# Autodesk Inventor assembly: 775pro_0_1-2inHex
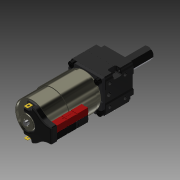
[picture p0: Inventor's stored thumbnail of the model, 180x180]
Saved by Autodesk Inventor 2021 (Build 250183000, 183)
## iProperties
Created: 2018-08-19
Part Number: 775pro_0_1-2inHex
Document SubType Name: Assembly
Designer: Rafi
Mass: 1123.04 g
Surface Area: 1203.25 cm^2
Volume: 285.054 cm^3
Density: 3.93975 g/cm^3
Author: Rafi
## Documents named in this file (7)
- D:\FIRST\FRC\1369\CollabPartsLib\Motors\Versaplanetary\VersaPlanetary\775pro, 0 Stages, 1-2in Hex Output.iam
- C:\Users\Cal\Desktop\GrabCAD\Meme-ataur 2020.5 Cadathon 9\Parts Library\Gearboxes\Planetary Gearboxes\V2 Stages\V2 Output Stage.iam
- C:\Users\Cal\Desktop\GrabCAD\Meme-ataur 2020.5 Cadathon 9\Parts Library\Gearboxes\Planetary Gearboxes\V2 Stages\V2 Input Stage.iam
- D:\FIRST\FRC\1369\CollabPartsLib\Motors\Versaplanetary\Screws\8-32 x 1.25in Screw.ipt
- D:\FIRST\FRC\1369\CollabPartsLib\Motors\Versaplanetary\V2 Stages\V2 Output Stage\VP V2 Output Stage 1-2in Hex.iam
- D:\FIRST\FRC\1369\CollabPartsLib\Motors\Versaplanetary\V2 Stages\V2 Input Stage\VP 775pro Input.iam
- D:\FIRST\FRC\1369\CollabPartsLib\Motors\Versaplanetary\VersaPlanetary.iam
## Components (4 placed, 3 different names)
1. VP V2 Output Stage 1-2in Hex:1 [sub-assembly] — 0StageBasicInputMate1, 0StageBasicInputMate2, 0StageBasicInputMate3
2. VP 775pro Input:1 [sub-assembly] — 0StageBasicInputMate1, 0StageBasicInputMate2, 0StageBasicInputMate3, Insert:12, Insert:13
3. 8-32 x 1.25in Screw:1 — Insert:12
4. 8-32 x 1.25in Screw:2 — Insert:13
## Relationships (5: Flush 2, Insert 2, Mate 1)
- 0StageBasicInputMate1 [Mate]: VP V2 Output Stage 1-2in Hex:1 ↔ VP 775pro Input:1
- 0StageBasicInputMate2 [Flush]: VP V2 Output Stage 1-2in Hex:1 ↔ VP 775pro Input:1
- 0StageBasicInputMate3 [Flush]: VP V2 Output Stage 1-2in Hex:1 ↔ VP 775pro Input:1
- Insert:12: VP 775pro Input:1 ↔ 8-32 x 1.25in Screw:1
- Insert:13: VP 775pro Input:1 ↔ 8-32 x 1.25in Screw:2
